# Autodesk Inventor assembly: Assembly1
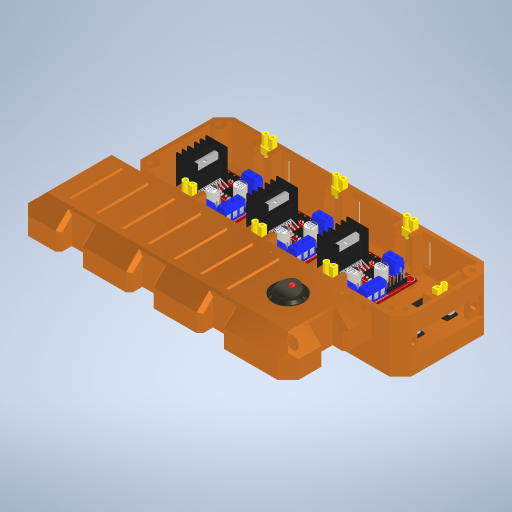
[picture p0: Inventor's stored thumbnail of the model, 512x512]
Saved by Autodesk Inventor 2024.2 (Build 282272000, 272)
## iProperties
Created: 2024-08-10
Part Number: Assembly1
Document SubType Name: Assembly
Designer: Admin
Author: Admin
## Documents named in this file (7)
- C:\Users\Admin\Documents\GitHub\ExplorateurErrant\Potencia\Assembly1.iam
- C:\Users\Admin\Documents\GitHub\ExplorateurErrant\Potencia\Sujecion.ipt
- C:\Users\Admin\Documents\GitHub\ExplorateurErrant\Potencia\H-Bridge\H-brug.ipt
- C:\Users\Admin\Documents\GitHub\ExplorateurErrant\Potencia\XT30-Female\XT30Female.ipt
- C:\Users\Admin\Documents\GitHub\ExplorateurErrant\Potencia\AmericanFuseHolder\AmericanFuseHolder\AmericanFuseHolder.ipt
- C:\Users\Admin\Documents\GitHub\ExplorateurErrant\Potencia\SwitchKCD\KCD1\KCD1.ipt
- C:\Users\Admin\Documents\GitHub\ExplorateurErrant\Potencia\TapaSujecion.ipt
## Components (14 placed, 6 different names)
1. Sujecion:1 — Mate:1, Mate:2, Mate:3, Mate:4, Mate:5, Mate:6, Mate:7, Mate:8, Mate:9, Mate:10, Mate:11, Mate:12, Mate:13, Mate:14, Mate:15, Mate:16, Mate:17, Mate:18, Mate:19, Mate:20, Mate:21, Mate:22, Mate:23, Mate:24, Mate:25, Mate:26, Mate:27, Mate:28, Mate:29, Mate:32, Mate:33, Mate:34
2. H-brug:1 — Mate:1, Mate:2, Mate:3
3. H-brug:2 — Mate:4, Mate:5, Mate:6
4. H-brug:3 — Mate:7, Mate:8, Mate:9
5. XT30Female:1 — Mate:10, Mate:11, Mate:12
6. XT30Female:2 — Mate:16, Mate:17, Mate:18
7. XT30Female:3 — Mate:25, Mate:26, Mate:27
8. XT30Female:4 — Mate:13, Mate:14, Mate:15
9. XT30Female:5 — Mate:19, Mate:20, Mate:21
10. XT30Female:6 — Mate:22, Mate:23, Mate:24
11. AmericanFuseHolder:1 — Mate:28, Mate:29
12. KCD1:1 — Mate:30, Mate:31
13. TapaSujecion:1 — Mate:30, Mate:31, Mate:32
14. XT30Female:7 — Mate:33, Mate:34
## Relationships (34: Mate 34)
- Mate:1: Sujecion:1 ↔ H-brug:1
- Mate:2: Sujecion:1 ↔ H-brug:1
- Mate:3: Sujecion:1 ↔ H-brug:1
- Mate:4: Sujecion:1 ↔ H-brug:2
- Mate:5: Sujecion:1 ↔ H-brug:2
- Mate:6: Sujecion:1 ↔ H-brug:2
- Mate:7: Sujecion:1 ↔ H-brug:3
- Mate:8: Sujecion:1 ↔ H-brug:3
- Mate:9: Sujecion:1 ↔ H-brug:3
- Mate:10: Sujecion:1 ↔ XT30Female:1
- Mate:11: Sujecion:1 ↔ XT30Female:1
- Mate:12: Sujecion:1 ↔ XT30Female:1
- Mate:13: Sujecion:1 ↔ XT30Female:4
- Mate:14: Sujecion:1 ↔ XT30Female:4
- Mate:15: Sujecion:1 ↔ XT30Female:4
- Mate:16: Sujecion:1 ↔ XT30Female:2
- Mate:17: Sujecion:1 ↔ XT30Female:2
- Mate:18: Sujecion:1 ↔ XT30Female:2
- Mate:19: Sujecion:1 ↔ XT30Female:5
- Mate:20: Sujecion:1 ↔ XT30Female:5
- Mate:21: Sujecion:1 ↔ XT30Female:5
- Mate:22: Sujecion:1 ↔ XT30Female:6
- Mate:23: Sujecion:1 ↔ XT30Female:6
- Mate:24: Sujecion:1 ↔ XT30Female:6
- Mate:25: Sujecion:1 ↔ XT30Female:3
- Mate:26: Sujecion:1 ↔ XT30Female:3
- Mate:27: Sujecion:1 ↔ XT30Female:3
- Mate:28: Sujecion:1 ↔ AmericanFuseHolder:1
- Mate:29: Sujecion:1 ↔ AmericanFuseHolder:1
- Mate:30: KCD1:1 ↔ TapaSujecion:1
- Mate:31: KCD1:1 ↔ TapaSujecion:1
- Mate:32: Sujecion:1 ↔ TapaSujecion:1
- Mate:33: Sujecion:1 ↔ XT30Female:7
- Mate:34: Sujecion:1 ↔ XT30Female:7
